# Autodesk Inventor assembly: cellSTORM_v4_flexure
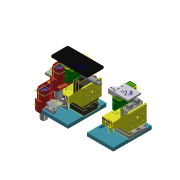
[picture p0: Inventor's stored thumbnail of the model, 180x180]
Saved by Autodesk Inventor 2019 (Build 230136000, 136)
## iProperties
Created: 2019-10-29
Part Number: cellSTORM_v4_flexure
Document SubType Name: Assembly
Designer: diederichbenedict
Author: diederichbenedict
## Documents named in this file (23)
- C:\Users\diederichbenedict\Dropbox\Dokumente\Promotion\PROJECTS\STORMoChip\GITHUB\CAD\Nanoscopy-on-the-cheap\Workspace\cellSTORM_v4_flexure.iam
- C:\Users\diederichbenedict\Dropbox\Dokumente\Promotion\PROJECTS\STORMoChip\GITHUB\CAD\Nanoscopy-on-the-cheap\Workspace\Assembly_Lasergroup_wPickup_v1.iam
- C:\Users\diederichbenedict\Dropbox\Dokumente\Promotion\PROJECTS\STORMoChip\GITHUB\CAD\Nanoscopy-on-the-cheap\Workspace\00_XY_stage-CHUO_SEIKI_LD-647-R1.iam
- C:\Users\diederichbenedict\Dropbox\Dokumente\Promotion\PROJECTS\STORMoChip\GITHUB\CAD\Nanoscopy-on-the-cheap\Workspace\02_Nanoscopy_Chip.ipt
- C:\Users\diederichbenedict\Dropbox\Dokumente\Promotion\PROJECTS\STORMoChip\GITHUB\CAD\Nanoscopy-on-the-cheap\Workspace\00_LASER_640nm.ipt
- C:\Users\diederichbenedict\Dropbox\Dokumente\Promotion\PROJECTS\STORMoChip\GITHUB\CAD\Nanoscopy-on-the-cheap\Workspace\00_KES400.iam
- C:\Users\diederichbenedict\Dropbox\Dokumente\Promotion\PROJECTS\STORMoChip\GITHUB\CAD\Nanoscopy-on-the-cheap\Workspace\00_Huawei_P20.ipt
- C:\Users\diederichbenedict\Dropbox\Dokumente\Promotion\PROJECTS\STORMoChip\GITHUB\CAD\Nanoscopy-on-the-cheap\Workspace\cellSTORM_Base_v0.ipt
- C:\Users\diederichbenedict\Dropbox\Dokumente\Promotion\PROJECTS\STORMoChip\GITHUB\CAD\Nanoscopy-on-the-cheap\Workspace\cellSTORM_Lasermount_v0.ipt
- C:\Users\diederichbenedict\Documents\Inventor\Content Center Files\R2019\en-US\DIN 912\DIN 912 - M3 x 0.5 x 25 x 18.ipt
- C:\Users\diederichbenedict\Dropbox\Dokumente\Promotion\PROJECTS\STORMoChip\GITHUB\CAD\Nanoscopy-on-the-cheap\Workspace\00_Ballmagnets_5mm.ipt
- C:\Users\diederichbenedict\Dropbox\Dokumente\Promotion\PROJECTS\STORMoChip\GITHUB\CAD\Nanoscopy-on-the-cheap\Workspace\00_Micrometer.ipt
- C:\Users\diederichbenedict\Dropbox\Dokumente\Promotion\PROJECTS\STORMoChip\GITHUB\CAD\Nanoscopy-on-the-cheap\Workspace\cellSTORM_Spacerring_ocular.ipt
- C:\Users\diederichbenedict\Dropbox\Dokumente\Promotion\PROJECTS\STORMoChip\GITHUB\CAD\Nanoscopy-on-the-cheap\Workspace\00_Blurayplayer_rod.ipt
- C:\Users\diederichbenedict\Dropbox\Dokumente\Promotion\PROJECTS\STORMoChip\GITHUB\CAD\Nanoscopy-on-the-cheap\Workspace\cellSTORM_cellphone_objectivelens_mount_flexure.ipt
- C:\Users\diederichbenedict\Dropbox\Dokumente\Promotion\PROJECTS\STORMoChip\GITHUB\CAD\Nanoscopy-on-the-cheap\Workspace\cellSTORM_cellphone_plate.ipt
- C:\Users\diederichbenedict\Dropbox\Dokumente\Promotion\PROJECTS\STORMoChip\GITHUB\CAD\Nanoscopy-on-the-cheap\Workspace\10_Filteslide_25mm.ipt
- C:\Users\diederichbenedict\Dropbox\Dokumente\Promotion\PROJECTS\STORMoChip\GITHUB\CAD\Nanoscopy-on-the-cheap\Workspace\cellSTORM_chip_Adapter_screws.ipt
- C:\Users\diederichbenedict\Dropbox\Dokumente\Promotion\PROJECTS\STORMoChip\GITHUB\CAD\Nanoscopy-on-the-cheap\Workspace\Assembly_Eyepiece_Folded_mirror_withfocus.iam
- C:\Users\diederichbenedict\Dropbox\Dokumente\Promotion\PROJECTS\STORMoChip\GITHUB\CAD\Nanoscopy-on-the-cheap\Workspace\cellSTORM_nickelplate.ipt
- C:\Users\diederichbenedict\Dropbox\Dokumente\Promotion\PROJECTS\STORMoChip\GITHUB\CAD\Nanoscopy-on-the-cheap\Workspace\cellSTORM_laserbeam.ipt
- C:\Users\diederichbenedict\Dropbox\Dokumente\Promotion\PROJECTS\STORMoChip\GITHUB\CAD\Nanoscopy-on-the-cheap\Workspace\00_XY_stage-Chinese_60x60.iam
- C:\Users\diederichbenedict\Dropbox\Dokumente\Promotion\PROJECTS\STORMoChip\GITHUB\CAD\Nanoscopy-on-the-cheap\Workspace\00_XY_stage-Chinese_60x60_R1.iam
## Components (37 placed, 22 different names)
1. Assembly_Lasergroup_wPickup_v1:1 [sub-assembly]
2. 00_KES400:1 [sub-assembly] — Mate:13, Mate:20, Mate:23, Mate:24
3. 00_Ballmagnets_5mm:2 — Mate:27
4. 00_Ballmagnets_5mm:5 — Mate:29
5. 00_Ballmagnets_5mm:6 — Mate:28
6. 00_Ballmagnets_5mm:7
7. cellSTORM_Base_v0:1 — Angle:16, Insert:32, Insert:33, Mate:26
8. cellSTORM_Lasermount_v0:1 — Insert:34, Insert:35, Angle:19, Insert:37, Insert:38, Mate:24, Insert:42, Insert:44
9. 00_LASER_640nm:1 — Mate:13, Angle:19, Insert:44, Flush:7
10. 02_Nanoscopy_Chip:2 — Mate:20, Angle:16, Mate:23, Mate:30
11. cellSTORM_Spacerring_ocular:1 — Insert:53
12. 00_XY_stage-CHUO_SEIKI_LD-647-R1:4 [sub-assembly] — Insert:37, Insert:38, Flush:2, Flush:3
13. 00_XY_stage-CHUO_SEIKI_LD-647-R1:5 [sub-assembly] — Insert:32, Insert:33, Insert:34, Insert:35
14. 00_Blurayplayer_rod:2 — Insert:42
15. cellSTORM_cellphone_objectivelens_mount_flexure:1 — Flush:2, Flush:3, Insert:51, Insert:52, Mate:25, Flush:6, Angle:20
16. cellSTORM_cellphone_plate:1 — Flush:6
17. cellSTORM_chip_Adapter_screws:1 — Mate:26, Insert:56, Insert:57, Insert:58
18. 00_Micrometer:1 — Insert:51
19. 00_Blurayplayer_rod:3 — Insert:52
20. Assembly_Eyepiece_Folded_mirror_withfocus:1 [sub-assembly] — Mate:25, Insert:53, Insert:54, Insert:55, Mate:31
21. 10_Filteslide_25mm:1 — Insert:54
22. 00_Huawei_P20:1 — Insert:55, Angle:20
23. DIN 912 - replaced by DIN EN ISO 4762 M3 x 25:7 — Insert:56, Mate:29
24. DIN 912 - replaced by DIN EN ISO 4762 M3 x 25:8 — Insert:57, Mate:28
25. DIN 912 - replaced by DIN EN ISO 4762 M3 x 25:9 — Insert:58, Mate:27
26. cellSTORM_nickelplate:1 — Mate:30
27. cellSTORM_laserbeam:1 — Flush:7
28. DIN 912 - replaced by DIN EN ISO 4762 M3 x 25:10 — Mate:31
29. 00_XY_stage-Chinese_60x60:1 [sub-assembly] — Mate:32, Flush:8, Mate:33, Insert:59
30. cellSTORM_Base_v0:2 — Mate:32, Flush:8, Mate:33
31. cellSTORM_Lasermount_v0:2 — Insert:59, Insert:60, Angle:21, Insert:61
32. 00_LASER_640nm:2 — Insert:60, Angle:21
33. cellSTORM_laserbeam:2
34. 00_XY_stage-Chinese_60x60_R1:1 [sub-assembly] — Insert:61, Insert:62
35. cellSTORM_cellphone_objectivelens_mount_flexure:2 — Insert:62
36. Assembly_Eyepiece_Folded_mirror_withfocus:2 [sub-assembly]
37. cellSTORM_cellphone_plate:2
## Relationships (42: Insert 20, Mate 13, Flush 5, Angle 4)
- Mate:13: 00_KES400:1 ↔ 00_LASER_640nm:1
- Mate:20: 00_KES400:1 ↔ 02_Nanoscopy_Chip:2
- Angle:16 (0 deg): cellSTORM_Base_v0:1 ↔ 02_Nanoscopy_Chip:2
- Mate:23 (2 mm): 00_KES400:1 ↔ 02_Nanoscopy_Chip:2
- Insert:32: cellSTORM_Base_v0:1 ↔ 00_XY_stage-CHUO_SEIKI_LD-647-R1:5
- Insert:33: cellSTORM_Base_v0:1 ↔ 00_XY_stage-CHUO_SEIKI_LD-647-R1:5
- Insert:34: cellSTORM_Lasermount_v0:1 ↔ 00_XY_stage-CHUO_SEIKI_LD-647-R1:5
- Insert:35: cellSTORM_Lasermount_v0:1 ↔ 00_XY_stage-CHUO_SEIKI_LD-647-R1:5
- Angle:19 (180 deg): cellSTORM_Lasermount_v0:1 ↔ 00_LASER_640nm:1
- Insert:37: cellSTORM_Lasermount_v0:1 ↔ 00_XY_stage-CHUO_SEIKI_LD-647-R1:4
- Insert:38: cellSTORM_Lasermount_v0:1 ↔ 00_XY_stage-CHUO_SEIKI_LD-647-R1:4
- Mate:24: 00_KES400:1 ↔ cellSTORM_Lasermount_v0:1
- Insert:42 (-6 mm): cellSTORM_Lasermount_v0:1 ↔ 00_Blurayplayer_rod:2
- Flush:2: 00_XY_stage-CHUO_SEIKI_LD-647-R1:4 ↔ cellSTORM_cellphone_objectivelens_mount_flexure:1
- Flush:3: 00_XY_stage-CHUO_SEIKI_LD-647-R1:4 ↔ cellSTORM_cellphone_objectivelens_mount_flexure:1
- Insert:44: cellSTORM_Lasermount_v0:1 ↔ 00_LASER_640nm:1
- Insert:51: cellSTORM_cellphone_objectivelens_mount_flexure:1 ↔ 00_Micrometer:1
- Insert:52: cellSTORM_cellphone_objectivelens_mount_flexure:1 ↔ 00_Blurayplayer_rod:3
- Mate:25: cellSTORM_cellphone_objectivelens_mount_flexure:1 ↔ Assembly_Eyepiece_Folded_mirror_withfocus:1
- Insert:53: cellSTORM_Spacerring_ocular:1 ↔ Assembly_Eyepiece_Folded_mirror_withfocus:1
- Insert:54: Assembly_Eyepiece_Folded_mirror_withfocus:1 ↔ 10_Filteslide_25mm:1
- Insert:55: Assembly_Eyepiece_Folded_mirror_withfocus:1 ↔ 00_Huawei_P20:1
- Mate:26: cellSTORM_Base_v0:1 ↔ cellSTORM_chip_Adapter_screws:1
- Insert:56 (7 mm): cellSTORM_chip_Adapter_screws:1 ↔ DIN 912 - replaced by DIN EN ISO 4762 M3 x 25:7
- Insert:57 (7 mm): cellSTORM_chip_Adapter_screws:1 ↔ DIN 912 - replaced by DIN EN ISO 4762 M3 x 25:8
- Insert:58 (7 mm): cellSTORM_chip_Adapter_screws:1 ↔ DIN 912 - replaced by DIN EN ISO 4762 M3 x 25:9
- Flush:6: cellSTORM_cellphone_objectivelens_mount_flexure:1 ↔ cellSTORM_cellphone_plate:1
- Mate:27: 00_Ballmagnets_5mm:2 ↔ DIN 912 - replaced by DIN EN ISO 4762 M3 x 25:9
- Mate:28: 00_Ballmagnets_5mm:6 ↔ DIN 912 - replaced by DIN EN ISO 4762 M3 x 25:8
- Mate:29: 00_Ballmagnets_5mm:5 ↔ DIN 912 - replaced by DIN EN ISO 4762 M3 x 25:7
- Mate:30: 02_Nanoscopy_Chip:2 ↔ cellSTORM_nickelplate:1
- Flush:7: 00_LASER_640nm:1 ↔ cellSTORM_laserbeam:1
- Mate:31: Assembly_Eyepiece_Folded_mirror_withfocus:1 ↔ DIN 912 - replaced by DIN EN ISO 4762 M3 x 25:10
- Angle:20 (180 deg): cellSTORM_cellphone_objectivelens_mount_flexure:1 ↔ 00_Huawei_P20:1
- Mate:32: 00_XY_stage-Chinese_60x60:1 ↔ cellSTORM_Base_v0:2
- Flush:8: 00_XY_stage-Chinese_60x60:1 ↔ cellSTORM_Base_v0:2
- Mate:33: 00_XY_stage-Chinese_60x60:1 ↔ cellSTORM_Base_v0:2
- Insert:59: 00_XY_stage-Chinese_60x60:1 ↔ cellSTORM_Lasermount_v0:2
- Insert:60: cellSTORM_Lasermount_v0:2 ↔ 00_LASER_640nm:2
- Angle:21 (180 deg): cellSTORM_Lasermount_v0:2 ↔ 00_LASER_640nm:2
- Insert:61: cellSTORM_Lasermount_v0:2 ↔ 00_XY_stage-Chinese_60x60_R1:1
- Insert:62: 00_XY_stage-Chinese_60x60_R1:1 ↔ cellSTORM_cellphone_objectivelens_mount_flexure:2
